# Autodesk Inventor assembly: Signal_tower
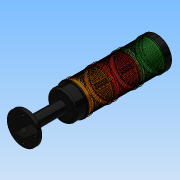
[picture p0: Inventor's stored thumbnail of the model, 180x180]
Saved by Autodesk Inventor 2017.3 (Build 213256000, 256)
## iProperties
Created: 2017-03-21
Material: Všeobecné
Document SubType Name: Assembly
Designer: CAD
Mass: 196.799 g
Surface Area: 1554.76 cm^2
Volume: 296.372 cm^3
Density: 0.664027 g/cm^3
Stock Number: SIEMENS
Part Number: Signal_tower
Hotovo: 0
Author: CAD
## Documents named in this file (6)
- C:\DATA\PC_CAD_alt_19082011\DATA\Privat\majak_CNC_stroj\Inv_2017\Signal_tower.iam
- C:\DATA\PC_CAD_alt_19082011\DATA\Privat\majak_CNC_stroj\Inv_2017\Signal_tower_A.ipt
- C:\DATA\PC_CAD_alt_19082011\DATA\Privat\majak_CNC_stroj\Inv_2017\Signal_tower_C.ipt
- C:\DATA\PC_CAD_alt_19082011\DATA\Privat\majak_CNC_stroj\Inv_2017\Signal_tower_B.ipt
- C:\DATA\PC_CAD_alt_19082011\DATA\Privat\majak_CNC_stroj\Inv_2017\Signal_tower_E.ipt
- C:\DATA\PC_CAD_alt_19082011\DATA\Privat\majak_CNC_stroj\Inv_2017\Signal_tower_D.ipt
## Components (5 placed, 5 different names)
1. Signal_tower_A:1 — Vložit:1
2. Signal_tower_B:1 — Vložit:1, Vložit:2
3. Signal_tower_C:2 — Vložit:2, Vložit:3
4. Signal_tower_D:1 — Vložit:3, Vložit:4
5. Signal_tower_E:1 — Vložit:4
## Relationships (4: Insert 4)
- Vložit:1 [Insert]: Signal_tower_A:1 ↔ Signal_tower_B:1
- Vložit:2 [Insert]: Signal_tower_B:1 ↔ Signal_tower_C:2
- Vložit:3 [Insert]: Signal_tower_C:2 ↔ Signal_tower_D:1
- Vložit:4 [Insert]: Signal_tower_D:1 ↔ Signal_tower_E:1
